# Autodesk Inventor assembly: EncoderPCBAssembly
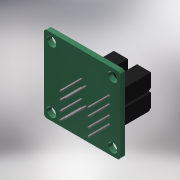
[picture p0: Inventor's stored thumbnail of the model, 180x180]
Saved by Autodesk Inventor 2018 (Build 220112000, 112)
## iProperties
Created: 2018-03-25
Part Number: EncoderPCBAssembly
Document SubType Name: Assembly
Designer: mansu
Author: mansu
## Documents named in this file (3)
- F:\OneDrive\Documents\2018 UBC\ELEC 391\Controller\cad\release\EncoderPCBAssembly.iam
- F:\OneDrive\Documents\2018 UBC\ELEC 391\Controller\cad\release\EncoderPCB.ipt
- F:\OneDrive\Documents\2018 UBC\ELEC 391\Controller\cad\release\GP1A52HRJ00F.ipt
## Components (3 placed, 2 different names)
1. EncoderPCB:1 — Flush:2, Mate:3, Flush:3
2. GP1A52HRJ00F:1 — Mate:1, Mate:2, Flush:1, Flush:2, Mate:3, Flush:3
3. GP1A52HRJ00F:2 — Mate:1, Mate:2, Flush:1
## Relationships (6: Mate 3, Flush 3)
- Mate:1: GP1A52HRJ00F:1 ↔ GP1A52HRJ00F:2
- Mate:2 (0.7 mm): GP1A52HRJ00F:1 ↔ GP1A52HRJ00F:2
- Flush:1: GP1A52HRJ00F:1 ↔ GP1A52HRJ00F:2
- Flush:2 (2 mm): EncoderPCB:1 ↔ GP1A52HRJ00F:1
- Mate:3 (0.5 mm): EncoderPCB:1 ↔ GP1A52HRJ00F:1
- Flush:3 (7 mm): EncoderPCB:1 ↔ GP1A52HRJ00F:1
